# Autodesk Inventor assembly: Bottom layer
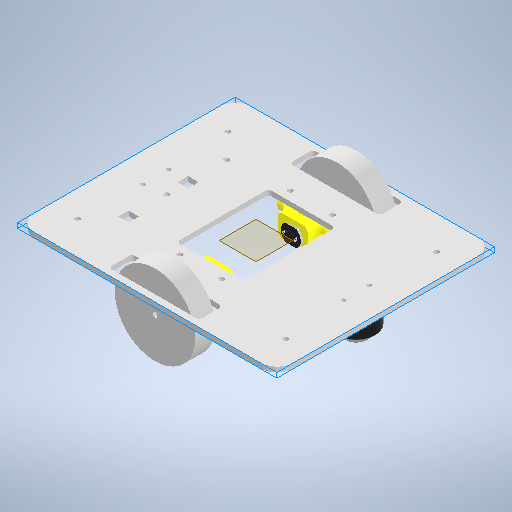
[picture p0: Inventor's stored thumbnail of the model, 512x512]
Saved by Autodesk Inventor 2025.1 (Build 291241000, 241)
## iProperties
Created: 2024-10-04
Part Number: Bottom layer
Document SubType Name: Assembly
Designer: bw1293
Author: bw1293
## Documents named in this file (4)
- C:\0_RDAC\Bw RDAC 1\Bottom layer.iam
- C:\0_RDAC\Bw RDAC 1\Bottom layer2.ipt
- C:\0_RDAC\Bw RDAC 1\Motor assembly.iam
- C:\0_RDAC\Bw RDAC 1\0.75in Ball Caster (Pololu).ipt
## Components (5 placed, 3 different names)
1. Bottom layer2:1 — Insert:1, Insert:2, Insert:3, Insert:4, Insert:5, Insert:6, Insert:7, Insert:8
2. Motor assembly:1 [sub-assembly] — Insert:3, Insert:4
3. Motor assembly:2 [sub-assembly] — Insert:1, Insert:2
4. 0.75in Ball Caster (Pololu):1 — Insert:5, Insert:6
5. 0.75in Ball Caster (Pololu):2 — Insert:7, Insert:8
## Relationships (8: Insert 8)
- Insert:1: Bottom layer2:1 ↔ Motor assembly:2
- Insert:2: Bottom layer2:1 ↔ Motor assembly:2
- Insert:3: Bottom layer2:1 ↔ Motor assembly:1
- Insert:4: Bottom layer2:1 ↔ Motor assembly:1
- Insert:5: Bottom layer2:1 ↔ 0.75in Ball Caster (Pololu):1
- Insert:6: Bottom layer2:1 ↔ 0.75in Ball Caster (Pololu):1
- Insert:7: Bottom layer2:1 ↔ 0.75in Ball Caster (Pololu):2
- Insert:8: Bottom layer2:1 ↔ 0.75in Ball Caster (Pololu):2
